# Autodesk Inventor assembly: FloatingIntake
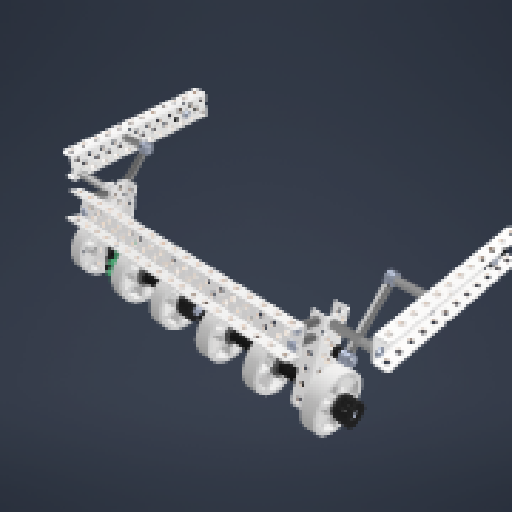
[picture p0: Inventor's stored thumbnail of the model, 512x512]
Saved by Autodesk Inventor 2023 (Build 270158000, 158)
## iProperties
Created: 2022-09-09
Part Number: FloatingIntake
Document SubType Name: Assembly
Designer: alex
Author: alex
## Documents named in this file (31)
- C:\Users\alex\Documents\GitHub\4067X_spin_up_cad\Mechanism\FloatingIntake.iam
- C:\Users\alex\Documents\GitHub\4067X_spin_up_cad\Library\Structure\C-Channels\Aluminum 1x2x1\Alu C 1x2x1x6.ipt
- C:\Users\alex\Documents\GitHub\4067X_spin_up_cad\Library\Motion\Shaft HS\Shaft HS\Shaft HS 12.0 in.ipt
- C:\Users\alex\Documents\GitHub\4067X_spin_up_cad\Library\Motion\Shaft HS\Shaft HS.ipt
- C:\Users\alex\Documents\GitHub\4067X_spin_up_cad\Library\Motion\Spacers\Spacer Nylon .375 OD.ipt
- C:\Users\alex\Documents\GitHub\4067X_spin_up_cad\Library\Motion\Shaft Collar with Set Screw.ipt
- C:\Users\alex\Documents\GitHub\4067X_spin_up_cad\WithAdapter2Inch.iam
- C:\Users\alex\Documents\GitHub\4067X_spin_up_cad\Library\Structure\Standoff\Standoff 2.00.ipt
- C:\Users\alex\Documents\GitHub\4067X_spin_up_cad\Library\Structure\Standoff.ipt
- C:\Users\alex\Documents\GitHub\4067X_spin_up_cad\Library\Structure\Standoff\Standoff .50.ipt
- C:\Users\alex\Documents\GitHub\4067X_spin_up_cad\Library\Structure\Standoff\Standoff 1.00.ipt
- C:\Users\alex\Documents\GitHub\4067X_spin_up_cad\Library\Motion\Shaft HS\HS Shaft Collar.ipt
- C:\Users\alex\Documents\GitHub\4067X_spin_up_cad\Library\Structure\Hardware\Screw Steel - Star.ipt
- C:\Users\alex\Documents\GitHub\4067X_spin_up_cad\Library\Structure\Hardware\Nut Keps.ipt
- C:\Users\alex\Documents\GitHub\4067X_spin_up_cad\Library\Structure\Hardware\Screw Steel - Star\SScrew Star Smooth .290.ipt
- C:\Users\alex\Documents\GitHub\4067X_spin_up_cad\Library\Structure\C-Channels\Aluminum 1x2x1\Alu C 1x2x1x12.ipt
- C:\Users\alex\Documents\GitHub\4067X_spin_up_cad\Library\Motion\1-Post Bearing Flat Hex Retainer.ipt
- C:\Users\alex\Documents\GitHub\4067X_spin_up_cad\Library\Structure\Hardware\Screw Steel - Star\SScrew Star Smooth .375.ipt
- C:\Users\alex\Documents\GitHub\4067X_spin_up_cad\Library\Structure\Hardware\Nut Nylock.ipt
- C:\Users\alex\Documents\GitHub\4067X_spin_up_cad\Library\Motion\Shaft HS\HS Bearing Flat.ipt
- C:\Users\alex\Documents\GitHub\4067X_spin_up_cad\Library\Motion\Shaft HS\HS Spacer\HSpacer .0625.ipt
- C:\Users\alex\Documents\GitHub\4067X_spin_up_cad\Library\Motion\Shaft HS\HS Spacer.ipt
- C:\Users\alex\Documents\GitHub\4067X_spin_up_cad\Library\Structure\Hardware\Screw Steel - Star\SScrew Star Smooth .500.ipt
- C:\Users\alex\Documents\GitHub\4067X_spin_up_cad\Library\Structure\Hardware\Nut Thin Nylock.ipt
- C:\Users\alex\Documents\GitHub\4067X_spin_up_cad\Library\Motion\Shaft HS\HS Spacer\HSpacer .5000.ipt
- C:\Users\alex\Documents\GitHub\4067X_spin_up_cad\Library\Motion\Sprockets\HS 12T Sprocket, No Insert.ipt
- C:\Users\alex\Documents\GitHub\4067X_spin_up_cad\Library\Motion\Shaft HS\HS Spacer\HSpacer .2500.ipt
- C:\Users\alex\Documents\GitHub\4067X_spin_up_cad\Library\Structure\C-Channels\Aluminum 1x2x1\Alu C 1x2x1x19.ipt
- C:\Users\alex\Documents\GitHub\4067X_spin_up_cad\Library\Structure\Standoff\Standoff .75.ipt
- C:\Users\alex\Documents\GitHub\4067X_spin_up_cad\Library\Motion\Spacers\Spacer Nylon .375 OD\NSpacer .375 OD x .250.ipt
- C:\Users\alex\Documents\GitHub\4067X_spin_up_cad\Library\Structure\Hardware\Screw Steel - Star\SScrew Star Smooth .750.ipt
## Components (77 placed, 25 different names)
1. Alu C 1x2x1x6:1 — Insert:64, Insert:67, Insert:80, Insert:81, Insert:94, Insert:98, Insert:102
2. Shaft HS 12.0 in:1
3. Shaft Collar with Set Screw:1 — Insert:97, Insert:101
4. Shaft Collar with Set Screw:2 — Insert:99, Insert:103
5. WithAdapter2Inch:1 [sub-assembly]
6. Standoff 2.00:1
7. HS Shaft Collar:1
8. SScrew Star Smooth .290:2
9. SScrew Star Smooth .290:3
10. Alu C 1x2x1x12:1 — Insert:92, Insert:96, Insert:100
11. 1-Post Bearing Flat Hex Retainer:1
12. SScrew Star Smooth .375:5
13. Nut Nylock:1
14. Alu C 1x2x1x12:2 — Insert:87, Insert:109, Insert:112
15. 1-Post Bearing Flat Hex Retainer:2
16. SScrew Star Smooth .375:6
17. Nut Nylock:2
18. Standoff 1.00:4 — Insert:88
19. Alu C 1x2x1x6:2 — Insert:72, Insert:73, Insert:78, Insert:79, Insert:110, Insert:111
20. HS Bearing Flat:1
21. HSpacer .0625:1
22. SScrew Star Smooth .500:10
23. Nut Thin Nylock:1
24. HSpacer .0625:2
25. WithAdapter2Inch:2 [sub-assembly]
26. HS Shaft Collar:2
27. HS Bearing Flat:2
28. Nut Thin Nylock:2
29. SScrew Star Smooth .500:11
30. WithAdapter2Inch:3 [sub-assembly]
31. HSpacer .5000:3
32. HSpacer .5000:4
33. WithAdapter2Inch:4 [sub-assembly]
34. WithAdapter2Inch:5 [sub-assembly]
35. HSpacer .5000:5
36. HSpacer .5000:6
37. WithAdapter2Inch:6 [sub-assembly]
38. HSpacer .5000:7
39. HSpacer .5000:8
40. HS 12T Sprocket, No Insert:1
41. HSpacer .5000:9
42. HSpacer .2500:10
43. HSpacer .2500:11
44. HS Shaft Collar:3
45. HS Shaft Collar:4
46. SScrew Star Smooth .290:12
47. SScrew Star Smooth .290:15 — Insert:64
48. Alu C 1x2x1x19:1 — Insert:74, Insert:75, Insert:76, Insert:77, Insert:82, Insert:83
49. SScrew Star Smooth .290:16 — Insert:67
50. SScrew Star Smooth .290:17 — Insert:72
51. SScrew Star Smooth .290:18 — Insert:73
52. SScrew Star Smooth .290:19 — Insert:74
53. SScrew Star Smooth .290:20 — Insert:75
54. SScrew Star Smooth .290:21 — Insert:76
55. SScrew Star Smooth .290:22 — Insert:77
56. Standoff .75:7 — Insert:78, Insert:83
57. Standoff .75:8 — Insert:79
58. Standoff .75:9 — Insert:80, Insert:82
59. Standoff .75:10 — Insert:81
60. Standoff .50:12 — Insert:87, Insert:88
61. Standoff .50:14 — Insert:92, Insert:93
62. Standoff 1.00:15 — Insert:93, Insert:94
63. Standoff 1.00:16 — Insert:96, Insert:97
64. NSpacer .375 OD x .250:5 — Insert:98, Insert:99
65. SScrew Star Smooth .290:23 — Insert:100
66. SScrew Star Smooth .375:24 — Insert:101
67. SScrew Star Smooth .750:25 — Insert:102
68. Nut Keps:5 — Insert:103
69. Shaft Collar with Set Screw:3
70. Shaft Collar with Set Screw:4
71. Standoff 2.00:17
72. Standoff 1.00:18 — Insert:109
73. NSpacer .375 OD x .250:6 — Insert:110
74. SScrew Star Smooth .375:26
75. Nut Keps:6
76. SScrew Star Smooth .750:27 — Insert:111
77. SScrew Star Smooth .290:28 — Insert:112
## Relationships (97: Insert 70, Mate 24, Flush 3)
- [Mate]: Alu C 1x2x1x6:1 ↔ Shaft HS 12.0 in:1
- [Mate]: Shaft Collar with Set Screw:1 ↔ Shaft Collar with Set Screw:2
- [Mate]: Shaft HS 12.0 in:1 ↔ WithAdapter2Inch:1
- [Mate]: Shaft HS 12.0 in:1 ↔ WithAdapter2Inch:1
- [Insert] (-0.3556 mm): Shaft Collar with Set Screw:2 ↔ Standoff 2.00:1
- [Mate] (-0.3556 mm): Shaft Collar with Set Screw:1 ↔ Standoff 2.00:1
- [Mate]: WithAdapter2Inch:1 ↔ HS Shaft Collar:1
- [Mate]: Shaft HS 12.0 in:1 ↔ HS Shaft Collar:1
- [Mate]: Shaft HS 12.0 in:1 ↔ HS Shaft Collar:1
- [Flush] (1.27 mm): Shaft HS 12.0 in:1 ↔ HS Shaft Collar:1
- [Insert]: Alu C 1x2x1x6:1 ↔ SScrew Star Smooth .290:2
- [Insert]: SScrew Star Smooth .290:3 ↔ Alu C 1x2x1x12:1
- [Insert]: Alu C 1x2x1x12:1 ↔ 1-Post Bearing Flat Hex Retainer:1
- [Mate]: Alu C 1x2x1x12:1 ↔ 1-Post Bearing Flat Hex Retainer:1
- [Insert]: Alu C 1x2x1x12:1 ↔ SScrew Star Smooth .375:5
- [Insert]: 1-Post Bearing Flat Hex Retainer:1 ↔ Nut Nylock:1
- [Insert]: Alu C 1x2x1x12:2 ↔ 1-Post Bearing Flat Hex Retainer:2
- [Mate]: Alu C 1x2x1x12:2 ↔ 1-Post Bearing Flat Hex Retainer:2
- [Insert]: Alu C 1x2x1x12:2 ↔ SScrew Star Smooth .375:6
- [Insert]: 1-Post Bearing Flat Hex Retainer:2 ↔ Nut Nylock:2
- [Flush]: Alu C 1x2x1x12:1 ↔ Alu C 1x2x1x12:2
- [Insert]: Standoff 1.00:4 ↔ Alu C 1x2x1x6:2
- [Insert]: Alu C 1x2x1x6:1 ↔ HS Bearing Flat:1
- [Mate]: Alu C 1x2x1x6:1 ↔ HS Bearing Flat:1
- [Mate]: Shaft HS 12.0 in:1 ↔ HSpacer .0625:1
- [Mate]: Alu C 1x2x1x6:1 ↔ HSpacer .0625:1
- [Mate]: WithAdapter2Inch:1 ↔ HSpacer .0625:1
- [Insert]: Alu C 1x2x1x6:1 ↔ SScrew Star Smooth .500:10
- [Insert]: HS Bearing Flat:1 ↔ Nut Thin Nylock:1
- [Mate]: Shaft HS 12.0 in:1 ↔ HSpacer .0625:2
- [Mate]: Alu C 1x2x1x6:2 ↔ HSpacer .0625:2
- [Mate]: Shaft HS 12.0 in:1 ↔ WithAdapter2Inch:2
- [Mate]: Shaft HS 12.0 in:1 ↔ WithAdapter2Inch:2
- [Mate]: HSpacer .0625:2 ↔ WithAdapter2Inch:2
- [Mate]: Shaft HS 12.0 in:1 ↔ HS Shaft Collar:2
- [Mate]: Shaft HS 12.0 in:1 ↔ HS Shaft Collar:2
- [Mate]: WithAdapter2Inch:2 ↔ HS Shaft Collar:2
- [Insert]: HS Bearing Flat:2 ↔ Nut Thin Nylock:2
- [Insert]: Alu C 1x2x1x6:2 ↔ HS Bearing Flat:2
- [Insert]: Alu C 1x2x1x6:2 ↔ HS Bearing Flat:2
- [Insert]: Alu C 1x2x1x6:2 ↔ SScrew Star Smooth .500:11
- [Insert]: WithAdapter2Inch:3 ↔ HSpacer .5000:3
- [Insert]: HSpacer .5000:5 ↔ HSpacer .5000:6
- [Insert]: HSpacer .5000:7 ↔ HSpacer .5000:8
- [Insert]: WithAdapter2Inch:6 ↔ HSpacer .5000:7
- [Insert]: HSpacer .5000:6 ↔ WithAdapter2Inch:6
- [Insert]: HS Bearing Flat:1 ↔ HSpacer .5000:8
- [Insert]: HS Bearing Flat:2 ↔ HSpacer .5000:9
- [Insert]: HS 12T Sprocket, No Insert:1 ↔ HSpacer .5000:9
- [Insert]: WithAdapter2Inch:3 ↔ HS 12T Sprocket, No Insert:1
- [Insert]: HSpacer .5000:3 ↔ HSpacer .5000:4
- [Insert]: HSpacer .5000:4 ↔ HSpacer .2500:10
- [Insert]: WithAdapter2Inch:4 ↔ HSpacer .2500:10
- [Insert]: HSpacer .5000:5 ↔ HSpacer .2500:11
- [Insert]: WithAdapter2Inch:5 ↔ HSpacer .2500:11
- [Insert]: WithAdapter2Inch:4 ↔ HS Shaft Collar:3
- [Insert]: WithAdapter2Inch:5 ↔ HS Shaft Collar:4
- [Flush]: Alu C 1x2x1x6:1 ↔ Alu C 1x2x1x6:2
- [Insert]: Alu C 1x2x1x6:2 ↔ SScrew Star Smooth .290:12
- Insert:64: Alu C 1x2x1x6:1 ↔ SScrew Star Smooth .290:15
- Insert:67: Alu C 1x2x1x6:1 ↔ SScrew Star Smooth .290:16
- Insert:72: Alu C 1x2x1x6:2 ↔ SScrew Star Smooth .290:17
- Insert:73: Alu C 1x2x1x6:2 ↔ SScrew Star Smooth .290:18
- Insert:74: Alu C 1x2x1x19:1 ↔ SScrew Star Smooth .290:19
- Insert:75: Alu C 1x2x1x19:1 ↔ SScrew Star Smooth .290:20
- Insert:76: Alu C 1x2x1x19:1 ↔ SScrew Star Smooth .290:21
- Insert:77: Alu C 1x2x1x19:1 ↔ SScrew Star Smooth .290:22
- Insert:78: Alu C 1x2x1x6:2 ↔ Standoff .75:7
- Insert:79: Alu C 1x2x1x6:2 ↔ Standoff .75:8
- Insert:80: Alu C 1x2x1x6:1 ↔ Standoff .75:9
- Insert:81: Alu C 1x2x1x6:1 ↔ Standoff .75:10
- Insert:82: Alu C 1x2x1x19:1 ↔ Standoff .75:9
- Insert:83: Alu C 1x2x1x19:1 ↔ Standoff .75:7
- Insert:87: Alu C 1x2x1x12:2 ↔ Standoff .50:12
- Insert:88: Standoff 1.00:4 ↔ Standoff .50:12
- Insert:92: Alu C 1x2x1x12:1 ↔ Standoff .50:14
- Insert:93: Standoff .50:14 ↔ Standoff 1.00:15
- Insert:94: Alu C 1x2x1x6:1 ↔ Standoff 1.00:15
- Insert:96: Alu C 1x2x1x12:1 ↔ Standoff 1.00:16
- Insert:97: Shaft Collar with Set Screw:1 ↔ Standoff 1.00:16
- Insert:98: Alu C 1x2x1x6:1 ↔ NSpacer .375 OD x .250:5
- Insert:99: Shaft Collar with Set Screw:2 ↔ NSpacer .375 OD x .250:5
- Insert:100: Alu C 1x2x1x12:1 ↔ SScrew Star Smooth .290:23
- Insert:101: Shaft Collar with Set Screw:1 ↔ SScrew Star Smooth .375:24
- Insert:102: Alu C 1x2x1x6:1 ↔ SScrew Star Smooth .750:25
- Insert:103: Shaft Collar with Set Screw:2 ↔ Nut Keps:5
- [Mate]: Shaft Collar with Set Screw:3 ↔ Shaft Collar with Set Screw:4
- [Insert] (-0.3556 mm): Shaft Collar with Set Screw:4 ↔ Standoff 2.00:17
- [Mate] (-0.3556 mm): Shaft Collar with Set Screw:3 ↔ Standoff 2.00:17
- [Insert]: Shaft Collar with Set Screw:3 ↔ Standoff 1.00:18
- [Insert]: Shaft Collar with Set Screw:4 ↔ NSpacer .375 OD x .250:6
- [Insert]: Shaft Collar with Set Screw:3 ↔ SScrew Star Smooth .375:26
- [Insert]: Shaft Collar with Set Screw:4 ↔ Nut Keps:6
- Insert:109: Alu C 1x2x1x12:2 ↔ Standoff 1.00:18
- Insert:110: Alu C 1x2x1x6:2 ↔ NSpacer .375 OD x .250:6
- Insert:111: Alu C 1x2x1x6:2 ↔ SScrew Star Smooth .750:27
- Insert:112: Alu C 1x2x1x12:2 ↔ SScrew Star Smooth .290:28
## Named parameters: d253_d244 = 0 mm, d265_d262_d260_d258 = 0 mm, d268_d262_d260_d258 = 0 mm, d269_d263_d261 = 0 mm, d205_d144 = 0 mm, d206_d145 = 0 mm, d207_d146 = 0 mm, d208_d147 = 0 mm, d149_d45 = 0 mm, d150_d48 = -0.3556 mm, d151_d49 = -0.3556 mm, d152_d138 = 0 mm, d153_d140 = 0 mm, d154_d142 = 0 mm, d155_d148 = 0 mm
